# Autodesk Inventor assembly: Chalk Applicator
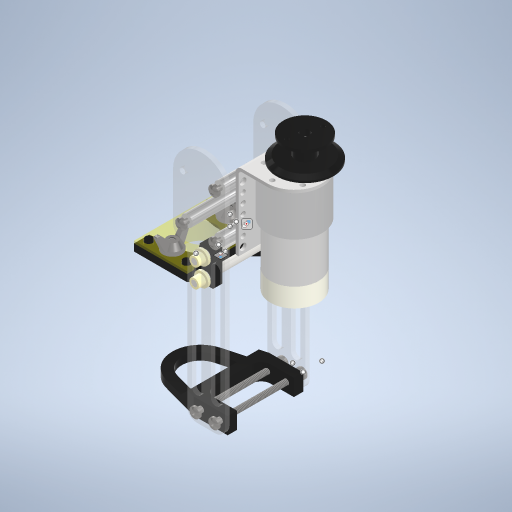
[picture p0: Inventor's stored thumbnail of the model, 512x512]
Saved by Autodesk Inventor 2024 (Build 280153000, 153)
## iProperties
Created: 2023-12-18
Part Number: Chalk Applicator
Document SubType Name: Assembly
Designer: greg
Author: greg
## Documents named in this file (13)
- C:\Users\greg\Documents\Inventor\Capstone\Chalk Applicator\Chalk Applicator.iam
- C:\Users\greg\Documents\Inventor\Capstone\Chalk Applicator\Cross Shaft.iam
- C:\Users\greg\Documents\Inventor\Capstone\Chalk Applicator\Side Plate.ipt
- C:\Users\greg\Documents\Inventor\Capstone\Chalk Applicator\Standoff.ipt
- C:\Users\greg\Documents\Inventor\Content Center Files\R2024\en-US\ANSI B18.6.3(60)\ANSI B18.6.3 - 6-32 UNC - 1.25(25).ipt
- C:\Users\greg\Documents\Inventor\Capstone\Chalk Applicator\Vince-Motor.iam
- C:\Users\greg\Documents\Inventor\Capstone\Chalk Applicator\Pulley.ipt
- C:\Users\greg\Documents\Inventor\Capstone\Chalk Applicator\Carriage.ipt
- C:\Users\greg\Documents\Inventor\Capstone\Chalk Applicator\Gripper.ipt
- C:\Users\greg\Documents\Inventor\Content Center Files\R2024\en-US\ANSI B18.6.3(24)\ANSI B18.6.3 - 10-24 UNC - 0.4375(4A).ipt
- C:\Users\greg\Documents\Inventor\Content Center Files\R2024\en-US\ANSI B18.22.1\ANSI B18.22.1 - No. 10 - Type A.ipt
- C:\Users\greg\Documents\Inventor\Content Center Files\R2024\en-US\ANSI B18.17(12)\ANSI B18.17 - No. 10 - 24 Light SeriesA (1).ipt
- C:\Users\greg\Documents\Inventor\Capstone\Chalk Applicator\Lower Guide.ipt
## Components (28 placed, 12 different names)
1. Side Plate:1 — Insert:6, Insert:7, Insert:8, Mate:21, Tangent:1, Mate:22, Tangent:2, Mate:27, Mate:39, Mate:40, Mate:41, Mate:42, Mate:43, Mate:44, Mate:45, Mate:46, Mate:47, Mate:48
2. Side Plate:2 — Insert:3, Insert:4, Insert:5, Mate:11, Mate:12, Mate:13, Mate:14, Mate:15, Mate:16, Mate:17, Mate:18, Mate:19, Mate:20, Mate:23, Mate:24, Flush:1
3. Cross Shaft:1 [sub-assembly] — Mate:22, Tangent:2, Mate:23, Mate:29
4. Cross Shaft:2 [sub-assembly] — Mate:21, Tangent:1, Mate:24, Mate:28, Mate:30
5. Standoff:3 — Insert:3, Insert:6, Tangent:3
6. Standoff:4 — Insert:4, Insert:8
7. Standoff:5 — Insert:5, Insert:7, Tangent:4, Tangent:5, Tangent:6
8. Square Recessed Pan Head Machine Screw - Type III - Inch (IFI) 6-32 UNC - 1.25:1 — Mate:39, Mate:40
9. Square Recessed Pan Head Machine Screw - Type III - Inch (IFI) 6-32 UNC - 1.25:6 — Mate:11, Mate:12
10. Square Recessed Pan Head Machine Screw - Type III - Inch (IFI) 6-32 UNC - 1.25:7 — Mate:13, Mate:14
11. Square Recessed Pan Head Machine Screw - Type III - Inch (IFI) 6-32 UNC - 1.25:8 — Mate:15, Mate:16
12. Square Recessed Pan Head Machine Screw - Type III - Inch (IFI) 6-32 UNC - 1.25:9 — Mate:17, Mate:18
13. Square Recessed Pan Head Machine Screw - Type III - Inch (IFI) 6-32 UNC - 1.25:10 — Mate:19, Mate:20
14. Vince-Motor:2 [sub-assembly] — Tangent:3, Tangent:4, Tangent:5, Tangent:6, Mate:25, Mate:26, Mate:27
15. Pulley:1 — Mate:25, Mate:26
16. Carriage:1 — Mate:28, Mate:29, Mate:30, Insert:11, Insert:12, Mate:31, Mate:32, Mate:33, Mate:34, Mate:35, Mate:37
17. Gripper:1 — Insert:11, Insert:12, Mate:36, Mate:38
18. Lower Guide:1 — Flush:1
19. Cross Recessed Pan Head Machine Screw - Type I - Inch No. 10 - 24 - 7/16:1 — Mate:31, Mate:32
20. Plain Washer (Inch) No. 10 - Type A:1 — Mate:35, Mate:36, Insert:13
21. Type A - Wing Nut - Inch No. 10 - 24 Light Series:1 — Insert:13
22. Cross Recessed Pan Head Machine Screw - Type I - Inch No. 10 - 24 - 7/16:2 — Mate:33, Mate:34
23. Plain Washer (Inch) No. 10 - Type A:2 — Mate:37, Mate:38, Insert:14
24. Type A - Wing Nut - Inch No. 10 - 24 Light Series:2 — Insert:14
25. Square Recessed Pan Head Machine Screw - Type III - Inch (IFI) 6-32 UNC - 1.25:11 — Mate:41, Mate:42
26. Square Recessed Pan Head Machine Screw - Type III - Inch (IFI) 6-32 UNC - 1.25:12 — Mate:43, Mate:44
27. Square Recessed Pan Head Machine Screw - Type III - Inch (IFI) 6-32 UNC - 1.25:13 — Mate:45, Mate:46
28. Square Recessed Pan Head Machine Screw - Type III - Inch (IFI) 6-32 UNC - 1.25:14 — Mate:47, Mate:48
## Relationships (55: Mate 38, Insert 10, Tangent 6, Flush 1)
- Insert:3: Side Plate:2 ↔ Standoff:3
- Insert:4: Side Plate:2 ↔ Standoff:4
- Insert:5: Side Plate:2 ↔ Standoff:5
- Insert:6: Side Plate:1 ↔ Standoff:3
- Insert:7: Side Plate:1 ↔ Standoff:5
- Insert:8: Side Plate:1 ↔ Standoff:4
- Mate:11: Side Plate:2 ↔ Square Recessed Pan Head Machine Screw - Type III - Inch (IFI) 6-32 UNC - 1.25:6
- Mate:12: Side Plate:2 ↔ Square Recessed Pan Head Machine Screw - Type III - Inch (IFI) 6-32 UNC - 1.25:6
- Mate:13: Side Plate:2 ↔ Square Recessed Pan Head Machine Screw - Type III - Inch (IFI) 6-32 UNC - 1.25:7
- Mate:14: Side Plate:2 ↔ Square Recessed Pan Head Machine Screw - Type III - Inch (IFI) 6-32 UNC - 1.25:7
- Mate:15: Side Plate:2 ↔ Square Recessed Pan Head Machine Screw - Type III - Inch (IFI) 6-32 UNC - 1.25:8
- Mate:16: Side Plate:2 ↔ Square Recessed Pan Head Machine Screw - Type III - Inch (IFI) 6-32 UNC - 1.25:8
- Mate:17: Side Plate:2 ↔ Square Recessed Pan Head Machine Screw - Type III - Inch (IFI) 6-32 UNC - 1.25:9
- Mate:18: Side Plate:2 ↔ Square Recessed Pan Head Machine Screw - Type III - Inch (IFI) 6-32 UNC - 1.25:9
- Mate:19: Side Plate:2 ↔ Square Recessed Pan Head Machine Screw - Type III - Inch (IFI) 6-32 UNC - 1.25:10
- Mate:20: Side Plate:2 ↔ Square Recessed Pan Head Machine Screw - Type III - Inch (IFI) 6-32 UNC - 1.25:10
- Mate:21: Side Plate:1 ↔ Cross Shaft:2
- Tangent:1: Side Plate:1 ↔ Cross Shaft:2
- Mate:22: Side Plate:1 ↔ Cross Shaft:1
- Tangent:2: Side Plate:1 ↔ Cross Shaft:1
- Mate:23: Side Plate:2 ↔ Cross Shaft:1
- Mate:24: Side Plate:2 ↔ Cross Shaft:2
- Tangent:3: Standoff:3 ↔ Vince-Motor:2
- Tangent:4: Standoff:5 ↔ Vince-Motor:2
- Tangent:5: Standoff:5 ↔ Vince-Motor:2
- Tangent:6: Standoff:5 ↔ Vince-Motor:2
- Mate:25: Vince-Motor:2 ↔ Pulley:1
- Mate:26: Vince-Motor:2 ↔ Pulley:1
- Mate:27 (6.6675 mm): Side Plate:1 ↔ Vince-Motor:2
- Mate:28: Cross Shaft:2 ↔ Carriage:1
- Mate:29: Cross Shaft:1 ↔ Carriage:1
- Mate:30 (1.5875 mm): Cross Shaft:2 ↔ Carriage:1
- Insert:11: Carriage:1 ↔ Gripper:1
- Insert:12: Carriage:1 ↔ Gripper:1
- Mate:31: Carriage:1 ↔ Cross Recessed Pan Head Machine Screw - Type I - Inch No. 10 - 24 - 7/16:1
- Mate:32: Carriage:1 ↔ Cross Recessed Pan Head Machine Screw - Type I - Inch No. 10 - 24 - 7/16:1
- Mate:33: Carriage:1 ↔ Cross Recessed Pan Head Machine Screw - Type I - Inch No. 10 - 24 - 7/16:2
- Mate:34: Carriage:1 ↔ Cross Recessed Pan Head Machine Screw - Type I - Inch No. 10 - 24 - 7/16:2
- Mate:35: Carriage:1 ↔ Plain Washer (Inch) No. 10 - Type A:1
- Mate:36: Gripper:1 ↔ Plain Washer (Inch) No. 10 - Type A:1
- Mate:37: Carriage:1 ↔ Plain Washer (Inch) No. 10 - Type A:2
- Mate:38: Gripper:1 ↔ Plain Washer (Inch) No. 10 - Type A:2
- Insert:13: Plain Washer (Inch) No. 10 - Type A:1 ↔ Type A - Wing Nut - Inch No. 10 - 24 Light Series:1
- Insert:14: Plain Washer (Inch) No. 10 - Type A:2 ↔ Type A - Wing Nut - Inch No. 10 - 24 Light Series:2
- Flush:1: Side Plate:2 ↔ Lower Guide:1
- Mate:39: Side Plate:1 ↔ Square Recessed Pan Head Machine Screw - Type III - Inch (IFI) 6-32 UNC - 1.25:1
- Mate:40: Side Plate:1 ↔ Square Recessed Pan Head Machine Screw - Type III - Inch (IFI) 6-32 UNC - 1.25:1
- Mate:41: Side Plate:1 ↔ Square Recessed Pan Head Machine Screw - Type III - Inch (IFI) 6-32 UNC - 1.25:11
- Mate:42: Side Plate:1 ↔ Square Recessed Pan Head Machine Screw - Type III - Inch (IFI) 6-32 UNC - 1.25:11
- Mate:43: Side Plate:1 ↔ Square Recessed Pan Head Machine Screw - Type III - Inch (IFI) 6-32 UNC - 1.25:12
- Mate:44: Side Plate:1 ↔ Square Recessed Pan Head Machine Screw - Type III - Inch (IFI) 6-32 UNC - 1.25:12
- Mate:45: Side Plate:1 ↔ Square Recessed Pan Head Machine Screw - Type III - Inch (IFI) 6-32 UNC - 1.25:13
- Mate:46: Side Plate:1 ↔ Square Recessed Pan Head Machine Screw - Type III - Inch (IFI) 6-32 UNC - 1.25:13
- Mate:47: Side Plate:1 ↔ Square Recessed Pan Head Machine Screw - Type III - Inch (IFI) 6-32 UNC - 1.25:14
- Mate:48: Side Plate:1 ↔ Square Recessed Pan Head Machine Screw - Type III - Inch (IFI) 6-32 UNC - 1.25:14
